# Autodesk Inventor assembly: Rover
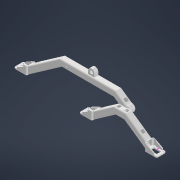
[picture p0: Inventor's stored thumbnail of the model, 180x180]
Saved by Autodesk Inventor 2021 (Build 250183000, 183)
## iProperties
Created: 2021-01-03
Part Number: Rover
Document SubType Name: Assembly
Designer: laure
Author: laure
## Documents named in this file (5)
- E:\Projects\Rover\Rover.iam
- E:\Projects\Rover\Rocker_hinten.ipt
- E:\Projects\Rover\Rocker_vorne.ipt
- E:\Projects\Rover\Servohalterung.ipt
- E:\Projects\Rover\Bogie.ipt
## Components (6 placed, 4 different names)
1. Fahrwerk_rocker_hinten:1 — Passend:3, Passend:4, Drehbar:1
2. Fahrwerk_rocker_vorne:1 — Passend:1, Passend:2, Passend:3, Passend:4
3. Servohalterung:1 — Passend:1, Passend:2
4. Servohalterung:2 — Passend:5, Passend:6
5. Servohalterung:3 — Passend:7, Passend:8
6. Fahrwerk_bogie:1 — Passend:5, Passend:6, Passend:7, Passend:8, Drehbar:1
## Relationships (9: Mate 8, RevoluteJoint 1)
- Passend:1 [Mate]: Fahrwerk_rocker_vorne:1 ↔ Servohalterung:1
- Passend:2 [Mate]: Fahrwerk_rocker_vorne:1 ↔ Servohalterung:1
- Passend:3 [Mate]: Fahrwerk_rocker_hinten:1 ↔ Fahrwerk_rocker_vorne:1
- Passend:4 [Mate]: Fahrwerk_rocker_hinten:1 ↔ Fahrwerk_rocker_vorne:1
- Passend:5 [Mate]: Servohalterung:2 ↔ Fahrwerk_bogie:1
- Passend:6 [Mate]: Servohalterung:2 ↔ Fahrwerk_bogie:1
- Passend:7 [Mate]: Servohalterung:3 ↔ Fahrwerk_bogie:1
- Passend:8 [Mate]: Servohalterung:3 ↔ Fahrwerk_bogie:1
- Drehbar:1 [RevoluteJoint]: Fahrwerk_rocker_hinten:1 ↔ Fahrwerk_bogie:1
